# Autodesk Inventor assembly: Gripper_Assembly
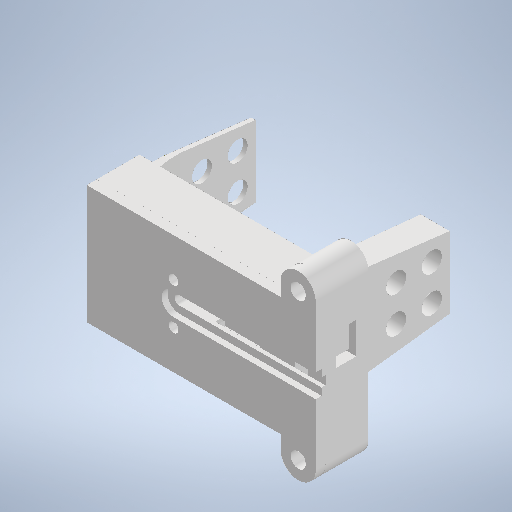
[picture p0: Inventor's stored thumbnail of the model, 512x512]
Saved by Autodesk Inventor 2025.1 (Build 291241000, 241)
## iProperties
Created: 2024-08-01
Part Number: Gripper_Assembly
Document SubType Name: Assembly
Designer: leonh
Author: leonh
## Documents named in this file (4)
- C:\Users\leonh\OneDrive\Dokumente\a_informatik\Inventor\Random\Gripper_Assembly.iam
- C:\Users\leonh\OneDrive\Dokumente\a_informatik\Inventor\Random\Rack_Gear_Gripper_V1.ipt
- C:\Users\leonh\OneDrive\Dokumente\a_informatik\Inventor\Random\Gripper_MountingBlock.ipt
- C:\Users\leonh\OneDrive\Dokumente\a_informatik\Inventor\Random\Gripper_MiddleMount_V1.ipt
## Components (4 placed, 3 different names)
1. Rack_Gear_Gripper_V1:1 — Slider:1, Symmetry:2
2. Rack_Gear_Gripper_V1:2 — Slider:1, Flush:1, Angle:1, Mate:1, Symmetry:2
3. Gripper_MountingBlock:1 — Flush:1, Angle:1, Mate:1, Mate:2, Angle:2, Insert:1, Mate:3
4. Gripper_MiddleMount_V1:1 — Mate:2, Angle:2, Insert:1
## Relationships (9: Mate 3, Angle 2, TranslationJoint 1, Flush 1, Symmetry 1, Insert 1)
- Slider:1 [TranslationJoint] (0.2 mm): Rack_Gear_Gripper_V1:1 ↔ Rack_Gear_Gripper_V1:2
- Flush:1: Rack_Gear_Gripper_V1:2 ↔ Gripper_MountingBlock:1
- Angle:1 (180 deg): Rack_Gear_Gripper_V1:2 ↔ Gripper_MountingBlock:1
- Mate:1 (0.1 mm): Rack_Gear_Gripper_V1:2 ↔ Gripper_MountingBlock:1
- Symmetry:2: Rack_Gear_Gripper_V1:1 ↔ Rack_Gear_Gripper_V1:2
- Mate:2: Gripper_MountingBlock:1 ↔ Gripper_MiddleMount_V1:1
- Angle:2 (0 deg): Gripper_MountingBlock:1 ↔ Gripper_MiddleMount_V1:1
- Insert:1: Gripper_MountingBlock:1 ↔ Gripper_MiddleMount_V1:1
- Mate:3: Gripper_MountingBlock:1
